# Autodesk Inventor assembly: KapalPembersihLaut
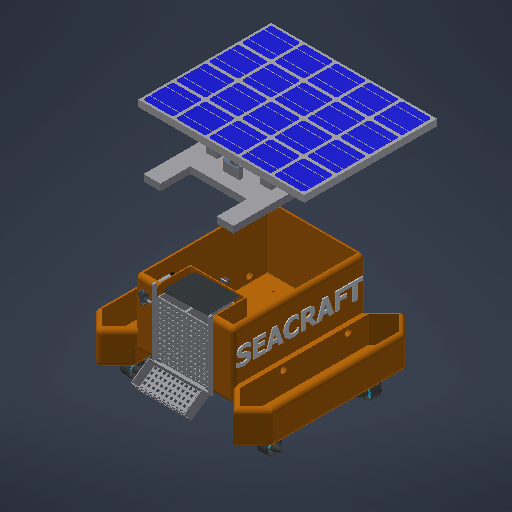
[picture p0: Inventor's stored thumbnail of the model, 512x512]
Saved by Autodesk Inventor 2026.2 (Build 302298000, 298)
## iProperties
Created: 2025-05-22
Part Number: KapalPembersihLaut
Document SubType Name: Assembly
Designer: hando
Author: hando
## Documents named in this file (20)
- D:\Data_Lokal\Kuliah\Tri Wahyu (22518241023)\Lomba Essay\Himpunan Administrasi Publik UNY\Design Kapal\KapalPembersihLaut.iam
- D:\Data_Lokal\Kuliah\Tri Wahyu (22518241023)\Lomba Essay\Himpunan Administrasi Publik UNY\Design Kapal\diamond-dynamics-thruster-1-2kg-1.snapshot.3\Thrusters v13\Thrusters v13\Thrusters v13.iam
- D:\Data_Lokal\Kuliah\Tri Wahyu (22518241023)\Lomba Essay\Himpunan Administrasi Publik UNY\Design Kapal\Base.ipt
- D:\Data_Lokal\Kuliah\Tri Wahyu (22518241023)\Lomba Essay\Himpunan Administrasi Publik UNY\Design Kapal\pg-36-dc-motor-1.snapshot.2\PG36.ipt
- D:\Data_Lokal\Kuliah\Tri Wahyu (22518241023)\Lomba Essay\Himpunan Administrasi Publik UNY\Design Kapal\bracket-pg36-1.snapshot.2\brecket encoder\brecket encoder\brecket encoder.ipt
- D:\Data_Lokal\Kuliah\Tri Wahyu (22518241023)\Lomba Essay\Himpunan Administrasi Publik UNY\Design Kapal\WadahSampah.ipt
- D:\Data_Lokal\Kuliah\Tri Wahyu (22518241023)\Lomba Essay\Himpunan Administrasi Publik UNY\Design Kapal\Solar panel.ipt
- D:\Data_Lokal\Kuliah\Tri Wahyu (22518241023)\Lomba Essay\Himpunan Administrasi Publik UNY\Design Kapal\Wadah+Solar.ipt
- D:\Data_Lokal\Kuliah\Tri Wahyu (22518241023)\Lomba Essay\Himpunan Administrasi Publik UNY\Design Kapal\Logitech c270 Assembly.iam
- D:\Data_Lokal\Kuliah\Tri Wahyu (22518241023)\Lomba Essay\Himpunan Administrasi Publik UNY\Design Kapal\Pengangkut.ipt
- D:\Data_Lokal\Kuliah\Tri Wahyu (22518241023)\Lomba Essay\Himpunan Administrasi Publik UNY\Design Kapal\KapalPembersihLaut\Design Accelerator\Bevel Gears1.iam
- D:\Data_Lokal\Kuliah\Tri Wahyu (22518241023)\Lomba Essay\Himpunan Administrasi Publik UNY\Design Kapal\KapalPembersihLaut\Design Accelerator\Bevel Gears2.iam
- D:\Data_Lokal\Kuliah\Tri Wahyu (22518241023)\Lomba Essay\Himpunan Administrasi Publik UNY\Design Kapal\Pemilah.ipt
- D:\Data_Lokal\Kuliah\Tri Wahyu (22518241023)\Lomba Essay\Himpunan Administrasi Publik UNY\Design Kapal\raspberry-pi-5-2.snapshot.8\RASPBERRY_PI_5\RASPBERRY_PI_5\RASPBERRY_PI_5.iam
- D:\Data_Lokal\Kuliah\Tri Wahyu (22518241023)\Lomba Essay\Himpunan Administrasi Publik UNY\Design Kapal\driverbtn v1.iam
- D:\Data_Lokal\Kuliah\Tri Wahyu (22518241023)\Lomba Essay\Himpunan Administrasi Publik UNY\Design Kapal\Pejal.ipt
- D:\Data_Lokal\Kuliah\Tri Wahyu (22518241023)\Lomba Essay\Himpunan Administrasi Publik UNY\Design Kapal\Jalur Pejal.ipt
- D:\Data_Lokal\Kuliah\Tri Wahyu (22518241023)\Lomba Essay\Himpunan Administrasi Publik UNY\Design Kapal\bevel-gear-217.snapshot.1\Bevel Gear 1\Bevel Gear 1\Bevel Gear 1.ipt
- D:\Data_Lokal\Kuliah\Tri Wahyu (22518241023)\Lomba Essay\Himpunan Administrasi Publik UNY\Design Kapal\Penyambung Jalur Pejal.ipt
- D:\Data_Lokal\Kuliah\Tri Wahyu (22518241023)\Lomba Essay\Himpunan Administrasi Publik UNY\Design Kapal\mg90-micro-servo-1.snapshot.5\MG90servo_assembly\MG90servo_assembly\MG90servo_assembly.iam
## Components (24 placed, 18 different names)
1. Thrusters v13:2 [sub-assembly] — Flush:7, Flush:8
2. Base:1 — Flush:1, Flush:2, Flush:3, Flush:4, Flush:5, Flush:6, Flush:7, Flush:8, Mate:8, Mate:9, Mate:10, Mate:11, Mate:15, Mate:16, Mate:19, Mate:20, Mate:23, Flush:14, Flush:15, Mate:25, Flush:17, Flush:18, Flush:19
3. Thrusters v13:3 [sub-assembly] — Flush:1, Flush:2
4. Thrusters v13:4 [sub-assembly] — Flush:3, Flush:4
5. Thrusters v13:5 [sub-assembly] — Flush:5, Flush:6
6. PG36:1 — Mate:3, Mate:4, Rotational:2
7. brecket encoder:1 — Mate:3, Mate:4, Mate:9, Mate:10, Mate:11
8. WadahSampah:1 — Mate:8, Flush:19
9. Solar panel:1 — Flush:11, Flush:12, Mate:17
10. Wadah+Solar:1 — Mate:15, Mate:16, Flush:11, Flush:12, Mate:17, Mate:18, Flush:13, Mate:21, Mate:22
11. Logitech c270 Assembly:1 [sub-assembly] — Mate:18, Flush:13
12. Pengangkut:1 — Rotational:1
13. Bevel Gears:1 [sub-assembly]
14. Bevel Gears:2 [sub-assembly]
15. Pemilah:1 — Mate:19, Mate:20, Mate:28
16. RASPBERRY_PI_5:1 [sub-assembly] — Mate:21
17. driverbtn v1:1 [sub-assembly] — Mate:22
18. Pejal:1 — Slider:1, Rotational:1
19. Jalur Pejal:1 — Mate:23, Flush:14, Flush:15, Slider:1
20. Jalur Pejal:2 — Mate:25, Flush:17, Flush:18
21. Bevel Gear 1:1 — Rotational:2
22. Bevel Gear 1:2 — Mate:26, Mate:27
23. Penyambung Jalur Pejal:1 — Mate:26, Mate:27
24. MG90servo_assembly:1 [sub-assembly] — Mate:28
## Relationships (38: Mate 19, Flush 16, RevoluteJoint 2, TranslationJoint 1)
- Flush:1 (5 mm): Base:1 ↔ Thrusters v13:3
- Flush:2 (3.5 mm): Base:1 ↔ Thrusters v13:3
- Flush:3 (3.5 mm): Base:1 ↔ Thrusters v13:4
- Flush:4 (5 mm): Base:1 ↔ Thrusters v13:4
- Flush:5 (5 mm): Base:1 ↔ Thrusters v13:5
- Flush:6 (3.5 mm): Base:1 ↔ Thrusters v13:5
- Flush:7 (5 mm): Thrusters v13:2 ↔ Base:1
- Flush:8 (3.5 mm): Thrusters v13:2 ↔ Base:1
- Mate:3: PG36:1 ↔ brecket encoder:1
- Mate:4: PG36:1 ↔ brecket encoder:1
- Mate:8: Base:1 ↔ WadahSampah:1
- Mate:9: Base:1 ↔ brecket encoder:1
- Mate:10: Base:1 ↔ brecket encoder:1
- Mate:11 (20 mm): Base:1 ↔ brecket encoder:1
- Mate:15: Base:1 ↔ Wadah+Solar:1
- Mate:16: Base:1 ↔ Wadah+Solar:1
- Flush:11 (-170 mm): Solar panel:1 ↔ Wadah+Solar:1
- Flush:12 (-190 mm): Solar panel:1 ↔ Wadah+Solar:1
- Mate:17: Solar panel:1 ↔ Wadah+Solar:1
- Mate:18 (50 mm): Wadah+Solar:1 ↔ Logitech c270 Assembly:1
- Flush:13 (125 mm): Wadah+Solar:1 ↔ Logitech c270 Assembly:1
- Mate:19: Base:1 ↔ Pemilah:1
- Mate:20 (5 mm): Base:1 ↔ Pemilah:1
- Mate:21: Wadah+Solar:1 ↔ RASPBERRY_PI_5:1
- Mate:22: Wadah+Solar:1 ↔ driverbtn v1:1
- Mate:23: Base:1 ↔ Jalur Pejal:1
- Flush:14: Base:1 ↔ Jalur Pejal:1
- Flush:15 (-10 mm): Base:1 ↔ Jalur Pejal:1
- Mate:25: Base:1 ↔ Jalur Pejal:2
- Flush:17 (-10 mm): Base:1 ↔ Jalur Pejal:2
- Flush:18: Base:1 ↔ Jalur Pejal:2
- Slider:1 [TranslationJoint] (125 mm): Pejal:1 ↔ Jalur Pejal:1
- Rotational:1 [RevoluteJoint] (-30 mm): Pengangkut:1 ↔ Pejal:1
- Rotational:2 [RevoluteJoint] (-10 mm): PG36:1 ↔ Bevel Gear 1:1
- Flush:19 (10 mm): Base:1 ↔ WadahSampah:1
- Mate:26: Bevel Gear 1:2 ↔ Penyambung Jalur Pejal:1
- Mate:27: Bevel Gear 1:2 ↔ Penyambung Jalur Pejal:1
- Mate:28: Pemilah:1 ↔ MG90servo_assembly:1
